# Autodesk Inventor assembly: Ensamble Actuador
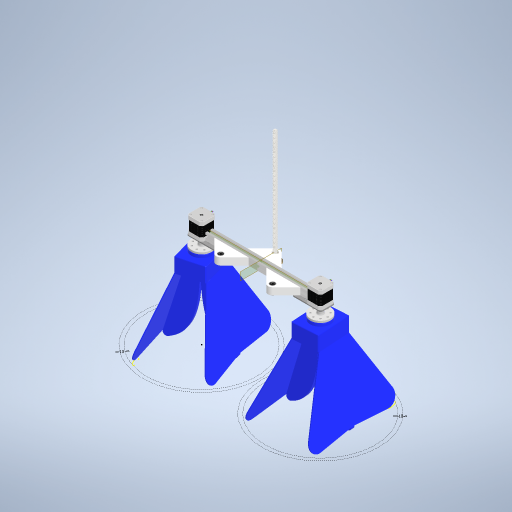
[picture p0: Inventor's stored thumbnail of the model, 512x512]
Saved by Autodesk Inventor 2023 (Build 270158000, 158)
## iProperties
Created: 2023-11-07
Part Number: Ensamble Actuador
Document SubType Name: Assembly
Designer: juanp
Author: juanp
## Documents named in this file (10)
- C:\Users\juanp\OneDrive - Universidad de los andes\Uniandes\GPR Portable\Actuador\Ensamble Actuador.iam
- C:\Users\juanp\OneDrive - Universidad de los andes\Uniandes\GPR Portable\Antenas\Antena PowerLog.ipt
- C:\Users\juanp\OneDrive - Universidad de los andes\Uniandes\GPR Portable\Actuador\Acople Antena - Motor.ipt
- C:\Users\juanp\OneDrive - Universidad de los andes\Uniandes\GPR Portable\Recursos\Movimiento\Motores\M1173041- NEMA 17.ipt
- C:\Users\juanp\OneDrive - Universidad de los andes\Uniandes\GPR Portable\Actuador\NEMA 17 Montura 2020.ipt
- C:\Users\juanp\OneDrive - Universidad de los andes\Uniandes\GPR Portable\Actuador\VSLOT 2020 actuador.ipt
- C:\Users\juanp\OneDrive - Universidad de los andes\Uniandes\GPR Portable\Actuador\Soporte Rieles - Antenas.ipt
- C:\Users\juanp\OneDrive - Universidad de los andes\Uniandes\GPR Portable\Actuador\Tornillo de potencia\Lead Screw.ipt
- C:\Users\juanp\OneDrive - Universidad de los andes\Uniandes\GPR Portable\Actuador\Tornillo de potencia\Nut.ipt
- C:\Users\juanp\OneDrive - Universidad de los andes\Uniandes\GPR Portable\Actuador\Rodamiento LM8UU\Lm8uu.iam
## Components (14 placed, 9 different names)
1. Antena PowerLog:1 — Mate:1, Flush:1, Mate:3, Mate:4
2. Antena PowerLog:2 — Mate:2, Flush:1, Mate:5
3. Acople Antena - Motor:1 — Flush:2, Mate:5, Mate:7, Mate:8
4. Acople Antena - Motor:2 — Flush:2, Mate:3, Mate:4, Mate:6
5. M1173041- NEMA 17:1 — Flush:3, Flush:4, Mate:6, Mate:9, Mate:14
6. M1173041- NEMA 17:2 — Flush:3, Flush:4, Mate:7, Mate:8, Mate:10, Mate:11, Mate:16
7. NEMA 17 Montura 2020:1 — Mate:9, Flush:5, Flush:6, Mate:12, Mate:15
8. NEMA 17 Montura 2020:2 — Mate:10, Flush:5, Mate:11, Flush:6, Mate:13
9. VSLOT 2020 actuador:1 — Mate:12, Mate:13, Mate:14, Mate:15, Mate:16, Mate:17, Mate:18, Mate:19, Mate:20, Mate:21, Flush:7
10. Soporte Rieles - Antenas:1 — Mate:20, Mate:21, Flush:7, Mate:22, Mate:23, Flush:9, Mate:24, Mate:25
11. Lead Screw:1 — Mate:26
12. Nut:1 — Mate:24, Mate:25, Mate:26
13. Lm8uu:1 [sub-assembly] — Flush:8, Mate:23, Flush:9
14. Lm8uu:2 [sub-assembly] — Flush:8, Mate:22
## Relationships (35: Mate 26, Flush 9)
- Mate:1: Antena PowerLog:1
- Mate:2: Antena PowerLog:2
- Flush:1: Antena PowerLog:1 ↔ Antena PowerLog:2
- Flush:2: Acople Antena - Motor:1 ↔ Acople Antena - Motor:2
- Mate:3: Antena PowerLog:1 ↔ Acople Antena - Motor:2
- Mate:4: Antena PowerLog:1 ↔ Acople Antena - Motor:2
- Mate:5: Antena PowerLog:2 ↔ Acople Antena - Motor:1
- Flush:3: M1173041- NEMA 17:1 ↔ M1173041- NEMA 17:2
- Flush:4: M1173041- NEMA 17:1 ↔ M1173041- NEMA 17:2
- Mate:6: Acople Antena - Motor:2 ↔ M1173041- NEMA 17:1
- Mate:7: Acople Antena - Motor:1 ↔ M1173041- NEMA 17:2
- Mate:8: Acople Antena - Motor:1 ↔ M1173041- NEMA 17:2
- Mate:9: M1173041- NEMA 17:1 ↔ NEMA 17 Montura 2020:1
- Mate:10: M1173041- NEMA 17:2 ↔ NEMA 17 Montura 2020:2
- Flush:5: NEMA 17 Montura 2020:1 ↔ NEMA 17 Montura 2020:2
- Mate:11: M1173041- NEMA 17:2 ↔ NEMA 17 Montura 2020:2
- Flush:6: NEMA 17 Montura 2020:1 ↔ NEMA 17 Montura 2020:2
- Mate:12: NEMA 17 Montura 2020:1 ↔ VSLOT 2020 actuador:1
- Mate:13: NEMA 17 Montura 2020:2 ↔ VSLOT 2020 actuador:1
- Mate:14: M1173041- NEMA 17:1 ↔ VSLOT 2020 actuador:1
- Mate:15: NEMA 17 Montura 2020:1 ↔ VSLOT 2020 actuador:1
- Mate:16: M1173041- NEMA 17:2 ↔ VSLOT 2020 actuador:1
- Mate:17: VSLOT 2020 actuador:1
- Mate:18: VSLOT 2020 actuador:1
- Mate:19: VSLOT 2020 actuador:1
- Mate:20: VSLOT 2020 actuador:1 ↔ Soporte Rieles - Antenas:1
- Mate:21: VSLOT 2020 actuador:1 ↔ Soporte Rieles - Antenas:1
- Flush:7: VSLOT 2020 actuador:1 ↔ Soporte Rieles - Antenas:1
- Flush:8: Lm8uu:1 ↔ Lm8uu:2
- Mate:22: Soporte Rieles - Antenas:1 ↔ Lm8uu:2
- Mate:23: Soporte Rieles - Antenas:1 ↔ Lm8uu:1
- Flush:9: Soporte Rieles - Antenas:1 ↔ Lm8uu:1
- Mate:24: Soporte Rieles - Antenas:1 ↔ Nut:1
- Mate:25: Soporte Rieles - Antenas:1 ↔ Nut:1
- Mate:26: Lead Screw:1 ↔ Nut:1
